# Autodesk Inventor assembly: KickerUnit
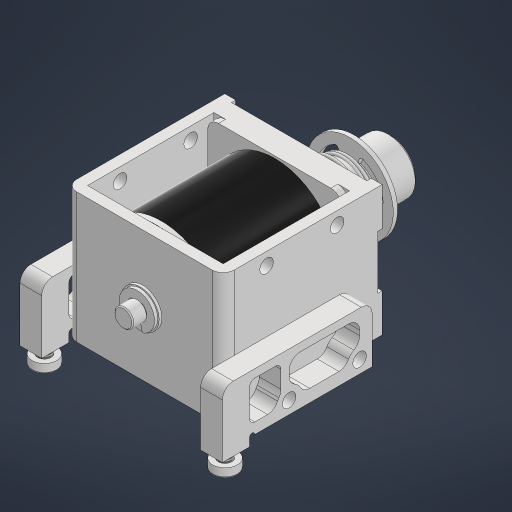
[picture p0: Inventor's stored thumbnail of the model, 512x512]
Saved by Autodesk Inventor 2024.2 (Build 282272000, 272)
## iProperties
Created: 2023-12-22
Part Number: KickerUnit
Document SubType Name: Assembly
Designer: Hanaoka
Author: Hanaoka
## Documents named in this file (5)
- G:\共有ドライブ\reRo\05_個人\hanaoka\inventor\KickerUnit\KickerUnit.iam
- G:\共有ドライブ\reRo\05_個人\hanaoka\inventor\KickerUnit\cb1029\cb1029.iam
- G:\共有ドライブ\reRo\05_個人\hanaoka\inventor\KickerUnit\SolenoidMount.ipt
- G:\共有ドライブ\reRo\05_個人\hanaoka\inventor\KickerUnit\SolenoidMount_MIR.ipt
- G:\共有ドライブ\reRo\05_個人\hanaoka\inventor\Screw\M2.6x8\M2.6x8.ipt
## Components (5 placed, 4 different names)
1. cb1029:1 [sub-assembly] — メイト:1, フラッシュ:1, 正接:1, フラッシュ:2, フラッシュ:3
2. SolenoidMount:1 — フラッシュ:2, フラッシュ:3, 挿入:2
3. SolenoidMount_MIR:1 — 挿入:1
4. M2.6x8:1 — 挿入:1
5. M2.6x8:2 — 挿入:2
## Relationships (7: Flush 3, Insert 2, Mate 1, Tangent 1)
- メイト:1 [Mate]: cb1029:1
- フラッシュ:1 [Flush]: cb1029:1
- 正接:1 [Tangent] (-1.75 mm): cb1029:1
- フラッシュ:2 [Flush]: cb1029:1 ↔ SolenoidMount:1
- フラッシュ:3 [Flush] (0.15 mm): cb1029:1 ↔ SolenoidMount:1
- 挿入:1 [Insert] (1.5 mm): SolenoidMount_MIR:1 ↔ M2.6x8:1
- 挿入:2 [Insert] (1.5 mm): SolenoidMount:1 ↔ M2.6x8:2
